# Autodesk Inventor assembly: new_shoulder2_elbow_strain_sensor_away
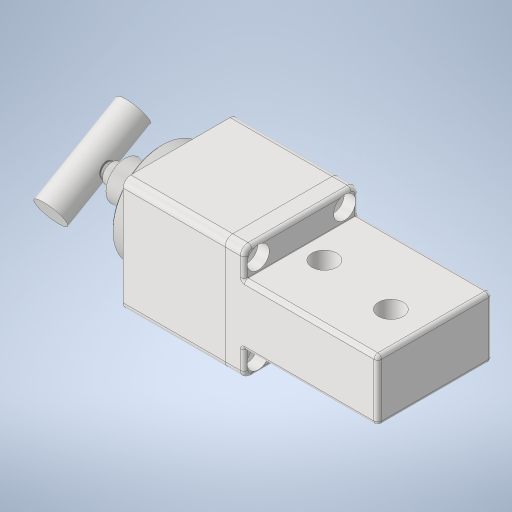
[picture p0: Inventor's stored thumbnail of the model, 512x512]
Saved by Autodesk Inventor 2024 (Build 280153000, 153)
## iProperties
Created: 2025-08-07
Part Number: new_shoulder2_elbow_strain_sensor_away
Document SubType Name: Assembly
Designer: HosodaLab2
Author: HosodaLab2
## Documents named in this file (6)
- C:\Users\HosodaLab2\OneDrive - Kyoto University\ドキュメント\Inventor\arm2\new_shoulder2_elbow_strain_sensor_away.iam
- C:\Users\HosodaLab2\OneDrive - Kyoto University\ドキュメント\Inventor\arm2\NewPart2.ipt
- C:\Users\HosodaLab2\OneDrive - Kyoto University\ドキュメント\Inventor\arm2\C-LHFR5.ipt
- C:\Users\HosodaLab2\OneDrive - Kyoto University\ドキュメント\Inventor\arm2\NewPart1.ipt
- C:\Users\HosodaLab2\OneDrive - Kyoto University\ドキュメント\Inventor\arm2\strain_sensor_jig.ipt
- C:\Users\HosodaLab2\OneDrive - Kyoto University\ドキュメント\Inventor\arm2\StrainSensor\SCLBRU5-38_0.iam
## Components (5 placed, 5 different names)
1. NewPart2:1 — 回転:1, 回転:2
2. C-LHFR5:1 — 回転:4, 回転:5, 円柱状:1
3. NewPart1:1 — 回転:1, 回転:2, 回転:4, 回転:5, フラッシュ:1
4. strain_sensor_jig:1 — 円柱状:2, フラッシュ:2
5. SCLBRU5-38_0:1 [sub-assembly] — 円柱状:1, フラッシュ:1, 円柱状:2, フラッシュ:2
## Relationships (8: RevoluteJoint 4, CylindricalJoint 2, Flush 2)
- 回転:1 [RevoluteJoint]: NewPart2:1 ↔ NewPart1:1
- 回転:2 [RevoluteJoint]: NewPart2:1 ↔ NewPart1:1
- 回転:4 [RevoluteJoint]: C-LHFR5:1 ↔ NewPart1:1
- 回転:5 [RevoluteJoint]: C-LHFR5:1 ↔ NewPart1:1
- 円柱状:1 [CylindricalJoint]: C-LHFR5:1 ↔ SCLBRU5-38_0:1
- フラッシュ:1 [Flush]: NewPart1:1 ↔ SCLBRU5-38_0:1
- 円柱状:2 [CylindricalJoint]: strain_sensor_jig:1 ↔ SCLBRU5-38_0:1
- フラッシュ:2 [Flush]: strain_sensor_jig:1 ↔ SCLBRU5-38_0:1
